# Autodesk Inventor assembly: AluminiumProfileAssembly
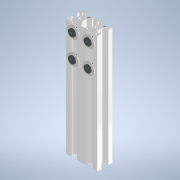
[picture p0: Inventor's stored thumbnail of the model, 180x180]
Saved by Autodesk Inventor 2022 (Build 260153000, 153)
## iProperties
Created: 2021-11-09
Part Number: AluminiumProfileAssembly
Document SubType Name: Assembly
Designer: JK
Author: JK
## Documents named in this file (5)
- C:\Users\JK\Documents\Inventor\UTM\AluminiumProfileAssembly.iam
- C:\Users\JK\Documents\Inventor\UTM\V-slot20×40x250mm.ipt
- C:\Users\JK\Documents\Inventor\UTM\M5 Washer.ipt
- C:\Users\JK\Documents\Inventor\UTM\PernoM5x25Plano.ipt
- C:\Users\JK\Documents\Inventor\UTM\TuercaTM5Perfil2020.ipt
## Components (13 placed, 4 different names)
1. V-slot20×40x250mm:1 — Coincidencia:3, Ángulo:1, Coincidencia:6, Coincidencia:7
2. PernoM5x25Plano:1 — Coincidencia:2, Coincidencia:3, Coincidencia:4, Coincidencia:5
3. M5 Washer:1 — Coincidencia:4, Coincidencia:5, Coincidencia:7
4. TuercaTM5Perfil2020:1 — Coincidencia:2, Ángulo:1, Coincidencia:6
5. PernoM5x25Plano:2
6. M5 Washer:2
7. TuercaTM5Perfil2020:2
8. PernoM5x25Plano:3
9. M5 Washer:3
10. TuercaTM5Perfil2020:3
11. PernoM5x25Plano:4
12. M5 Washer:4
13. TuercaTM5Perfil2020:4
## Component patterns: (4 elements, first: PernoM5x25Plano:1 + M5 Washer:1 + TuercaTM5Perfil2020:1)
## Relationships (7: Mate 6, Angle 1)
- Coincidencia:2 [Mate]: PernoM5x25Plano:1 ↔ TuercaTM5Perfil2020:1
- Coincidencia:3 [Mate]: V-slot20×40x250mm:1 ↔ PernoM5x25Plano:1
- Ángulo:1 [Angle] (0 deg): V-slot20×40x250mm:1 ↔ TuercaTM5Perfil2020:1
- Coincidencia:4 [Mate]: PernoM5x25Plano:1 ↔ M5 Washer:1
- Coincidencia:5 [Mate]: PernoM5x25Plano:1 ↔ M5 Washer:1
- Coincidencia:6 [Mate] (0.5 mm): V-slot20×40x250mm:1 ↔ TuercaTM5Perfil2020:1
- Coincidencia:7 [Mate]: V-slot20×40x250mm:1 ↔ M5 Washer:1
